# Autodesk Inventor assembly: base
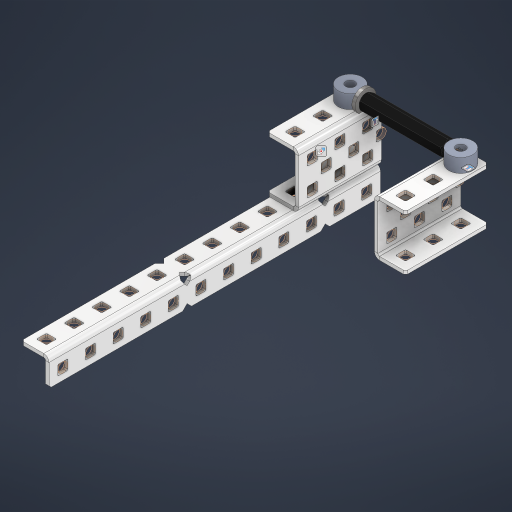
[picture p0: Inventor's stored thumbnail of the model, 512x512]
Saved by Autodesk Inventor 2024 (Build 280153000, 153)
## iProperties
Created: 2023-10-22
Part Number: base
Document SubType Name: Assembly
Designer: Averey Ku
Author: Averey Ku
## Documents named in this file (8)
- D:\vex_robotics\hardware\cad\spades_v0.1\intake\base.iam
- D:\vex_robotics\hardware\cad\VEX-CAD-Inventor-1.41\Structure\C Channel\Aluminum 1x2x1\Alu C 1x2x1x3.ipt
- D:\vex_robotics\hardware\cad\VEX-CAD-Inventor-1.41\Motion\Shaft LS\Shaft Collar ipts\Shaft Collar No Screw.ipt
- D:\vex_robotics\hardware\cad\VEX-CAD-Inventor-1.41\Structure\Standoff.ipt
- D:\vex_robotics\hardware\cad\VEX-CAD-Inventor-1.41\Motion\Spacers\Washer Steel\SWasher .375 OD x .062500.ipt
- D:\vex_robotics\hardware\cad\VEX-CAD-Inventor-1.41\Motion\Spacers\Washer Steel.ipt
- D:\vex_robotics\hardware\cad\VEX-CAD-Inventor-1.41\Structure\Angle\Aluminum 1x1\Alu Angle 1x1x12.ipt
- D:\vex_robotics\hardware\cad\VEX-CAD-Inventor-1.41\Structure\Standoff\Standoff 1.50.ipt
## Components (7 placed, 5 different names)
1. Alu C 1x2x1x3:1 — Insert:1, Mate:1, Insert:2, Insert:6, Mate:3
2. Alu C 1x2x1x3:2 — Insert:1, Mate:1, Insert:3
3. Shaft Collar No Screw:1 — Insert:2, Angle:1, Mate:2, Insert:5
4. Shaft Collar No Screw:2 — Insert:3, Angle:1, Mate:2
5. SWasher .375 OD x .062500:1 — Insert:5, Insert:7
6. Alu Angle 1x1x12:1 — Insert:6, Mate:3
7. Standoff 1.50:1 — Insert:7
## Relationships (10: Insert 6, Mate 3, Angle 1)
- Insert:1 (34.925 mm): Alu C 1x2x1x3:1 ↔ Alu C 1x2x1x3:2
- Mate:1: Alu C 1x2x1x3:1 ↔ Alu C 1x2x1x3:2
- Insert:2: Alu C 1x2x1x3:1 ↔ Shaft Collar No Screw:1
- Insert:3: Alu C 1x2x1x3:2 ↔ Shaft Collar No Screw:2
- Angle:1 (0 deg): Shaft Collar No Screw:1 ↔ Shaft Collar No Screw:2
- Mate:2: Shaft Collar No Screw:1 ↔ Shaft Collar No Screw:2
- Insert:5: Shaft Collar No Screw:1 ↔ SWasher .375 OD x .062500:1
- Insert:6: Alu C 1x2x1x3:1 ↔ Alu Angle 1x1x12:1
- Mate:3: Alu C 1x2x1x3:1 ↔ Alu Angle 1x1x12:1
- Insert:7: SWasher .375 OD x .062500:1 ↔ Standoff 1.50:1
